# Autodesk Inventor assembly: Arduino_zlozenie
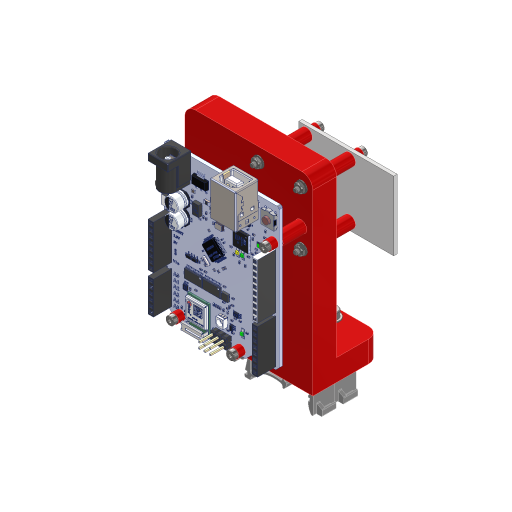
[picture p0: Inventor's stored thumbnail of the model, 512x512]
Saved by Autodesk Inventor 2024.3 (Build 283343000, 343)
## iProperties
Created: 2025-06-18
Part Number: Arduino_zlozenie
Document SubType Name: Assembly
Designer: MPA
Author: MPA
## Documents named in this file (13)
- C:\MPA - shortPath\magisterka\V3\Workspace\Arduino_zlozenie.iam
- C:\MPA - shortPath\magisterka\V3\Workspace\Zakupowe\arduino\Arduino UNO Wifi\Arduino UNO Wifi\Arduino UNO Wifi.ipt
- C:\MPA - shortPath\magisterka\V3\Workspace\MontazWszafie\Arduino-cz1.ipt
- C:\MPA - shortPath\magisterka\V3\Workspace\MontazWszafie\Arduino-cz2.ipt
- C:\MPA - shortPath\magisterka\V3\Workspace\MontazWszafie\2698103\2698103\NS_35_7.5_PERF_18X5.2_2000MM-Select.ipt
- C:\MPA - shortPath\magisterka\V3\Workspace\MontazWszafie\1201578_PHOENIX\1201578_PHOENIX\1201578_PHOENIX.ipt
- C:\MPA - shortPath\magisterka\V3\Workspace\MontazWszafie\Uchwyt_arduino.ipt
- C:\MPA - shortPath\magisterka\V3\Workspace\cc\en-US\Copy of DIN 912 - replaced by DIN EN ISO 4762\Copy of DIN 912 - M2 x 0,4 x 30 x 19.ipt
- C:\MPA - shortPath\magisterka\V3\Workspace\cc\en-US\DIN 125-1  A\DIN 125 - A 2,2.ipt
- C:\MPA - shortPath\magisterka\V3\Workspace\cc\en-US\DIN 934\DIN 934 - M2 x 0,4.ipt
- C:\MPA - shortPath\magisterka\V3\Workspace\cc\en-US\DIN 125-1  A\DIN 125 - A 3,2.ipt
- C:\MPA - shortPath\magisterka\V3\Workspace\cc\en-US\Copy of DIN 912 - replaced by DIN EN ISO 4762\Copy of DIN 912 - M3 x 0,5 x 16 x 14,75.ipt
- C:\MPA - shortPath\magisterka\V3\Workspace\DFR-08104.ipt
## Components (75 placed, 12 different names)
1. Arduino UNO Wifi:1 — Insert:1, Insert:2, Insert:3, Insert:4, Insert:5, Insert:6, Insert:7, Insert:8
2. Arduino-cz1:1 — Insert:2
3. Arduino-cz1:2 — Insert:3, Mate:5, Mate:7, Mate:9, Mate:11
4. Arduino-cz1:3 — Insert:4
5. Arduino-cz1:4 — Insert:1
6. Arduino-cz2:1 — Insert:5, Flush:9
7. Arduino-cz2:2 — Insert:6
8. Arduino-cz2:3 — Insert:7
9. Arduino-cz2:4 — Insert:8
10. NS_35_7.5_PERF_18X5.2_2000MM-Select:1 — Flush:4, Flush:5, Flush:6, Mate:2, Mate:3, Flush:11
11. 1201578_PHOENIX:1 — Flush:7, Flush:8, Mate:1, Mate:2
12. 1201578_PHOENIX:2 — Flush:7, Flush:8, Mate:1, Mate:3, Mate:20, Flush:10
13. Uchwyt_arduino:1 — Flush:9, Mate:4, Mate:6, Mate:8, Mate:10, Mate:12, Mate:13, Mate:14, Mate:15, Mate:16, Mate:17, Mate:18, Mate:19, Mate:20, Flush:10, Flush:11, Mate:21, Mate:22, Mate:23, Mate:24, Mate:25, Mate:26, Mate:27, Mate:28, Insert:33, Insert:34, Mate:29, Mate:30, Mate:31, Mate:33, Mate:35, Mate:37, Mate:39, Mate:41, Mate:43, Mate:45, Mate:47, Mate:48, Mate:49, Mate:50, Mate:51, Mate:52, Mate:53, Mate:54, Mate:55, Mate:56, Mate:57, Mate:58, Mate:59, Mate:60, Mate:61, Mate:62
14. Copy of DIN 912 - replaced by DIN EN ISO 4762 M2 x 30:1 — Mate:4, Mate:5
15. DIN 125-1 A A 2,2:1 — Mate:12, Mate:13, Insert:9
16. DIN 934 - replaced by DIN EN 24032/28673/28674 M2:1 — Insert:9
17. Copy of DIN 912 - replaced by DIN EN ISO 4762 M2 x 30:2 — Mate:6, Mate:7
18. Copy of DIN 912 - replaced by DIN EN ISO 4762 M2 x 30:3 — Mate:8, Mate:9
19. Copy of DIN 912 - replaced by DIN EN ISO 4762 M2 x 30:4 — Mate:10, Mate:11
20. DIN 125-1 A A 2,2:2 — Mate:14, Mate:15, Insert:10
21. DIN 125-1 A A 2,2:3 — Mate:16, Mate:17, Insert:11
22. DIN 125-1 A A 2,2:4 — Mate:18, Mate:19, Insert:12
23. DIN 934 - replaced by DIN EN 24032/28673/28674 M2:2 — Insert:10
24. DIN 934 - replaced by DIN EN 24032/28673/28674 M2:3 — Insert:11
25. DIN 934 - replaced by DIN EN 24032/28673/28674 M2:4 — Insert:12
26. DIN 125-1 A A 3,2:1 — Mate:21, Mate:22, Insert:13
27. Copy of DIN 912 - replaced by DIN EN ISO 4762 M3 x 16:1 — Insert:13
28. DIN 125-1 A A 3,2:2 — Mate:23, Mate:24, Insert:14
29. DIN 125-1 A A 3,2:3 — Mate:25, Mate:26, Insert:15
30. DIN 125-1 A A 3,2:4 — Mate:27, Mate:28, Insert:16
31. Copy of DIN 912 - replaced by DIN EN ISO 4762 M3 x 16:2 — Insert:14
32. Copy of DIN 912 - replaced by DIN EN ISO 4762 M3 x 16:3 — Insert:15
33. Copy of DIN 912 - replaced by DIN EN ISO 4762 M3 x 16:4 — Insert:16
34. Arduino-cz2:6 — Insert:17, Mate:30
35. Arduino-cz2:7 — Insert:19
36. Arduino-cz2:8 — Insert:18, Insert:33
37. Arduino-cz2:9 — Insert:20
38. DFR-08104:2 — Insert:17, Insert:18, Insert:19, Insert:20, Insert:21, Insert:22, Insert:23, Insert:24
39. Arduino-cz1:5 — Insert:21
40. Arduino-cz1:6 — Insert:23
41. Arduino-cz1:7 — Insert:24
42. Arduino-cz1:8 — Insert:22
43. Arduino-cz2:10 — Insert:34
44. Arduino-cz2:11
45. Arduino-cz2:12 — Mate:29
46. Arduino-cz2:13
47. DFR-08104:3
48. Arduino-cz1:9
49. Arduino-cz1:10
50. Arduino-cz1:11 — Mate:32, Mate:34, Mate:36, Mate:38, Mate:40, Mate:42, Mate:44, Mate:46
51. Arduino-cz1:12
52. Copy of DIN 912 - replaced by DIN EN ISO 4762 M2 x 30:5 — Mate:31, Mate:32
53. DIN 125-1 A A 2,2:5 — Mate:47, Mate:48, Insert:35
54. DIN 934 - replaced by DIN EN 24032/28673/28674 M2:5 — Insert:35
55. Copy of DIN 912 - replaced by DIN EN ISO 4762 M2 x 30:6 — Mate:33, Mate:34
56. Copy of DIN 912 - replaced by DIN EN ISO 4762 M2 x 30:7 — Mate:35, Mate:36
57. Copy of DIN 912 - replaced by DIN EN ISO 4762 M2 x 30:8 — Mate:37, Mate:38
58. Copy of DIN 912 - replaced by DIN EN ISO 4762 M2 x 30:9 — Mate:39, Mate:40
59. Copy of DIN 912 - replaced by DIN EN ISO 4762 M2 x 30:10 — Mate:41, Mate:42
60. Copy of DIN 912 - replaced by DIN EN ISO 4762 M2 x 30:11 — Mate:43, Mate:44
61. Copy of DIN 912 - replaced by DIN EN ISO 4762 M2 x 30:12 — Mate:45, Mate:46
62. DIN 125-1 A A 2,2:6 — Mate:49, Mate:50, Insert:36
63. DIN 125-1 A A 2,2:7 — Mate:51, Mate:52, Insert:37
64. DIN 125-1 A A 2,2:8 — Mate:53, Mate:54, Insert:38
65. DIN 125-1 A A 2,2:9 — Mate:55, Mate:56, Insert:39
66. DIN 125-1 A A 2,2:10 — Mate:57, Mate:58, Insert:40
67. DIN 125-1 A A 2,2:11 — Mate:59, Mate:60, Insert:41
68. DIN 125-1 A A 2,2:12 — Mate:61, Mate:62, Insert:42
69. DIN 934 - replaced by DIN EN 24032/28673/28674 M2:6 — Insert:36
70. DIN 934 - replaced by DIN EN 24032/28673/28674 M2:7 — Insert:37
71. DIN 934 - replaced by DIN EN 24032/28673/28674 M2:8 — Insert:38
72. DIN 934 - replaced by DIN EN 24032/28673/28674 M2:9 — Insert:39
73. DIN 934 - replaced by DIN EN 24032/28673/28674 M2:10 — Insert:40
74. DIN 934 - replaced by DIN EN 24032/28673/28674 M2:11 — Insert:41
75. DIN 934 - replaced by DIN EN 24032/28673/28674 M2:12 — Insert:42
## Relationships (112: Mate 62, Insert 42, Flush 8)
- Insert:1: Arduino UNO Wifi:1 ↔ Arduino-cz1:4
- Insert:2: Arduino UNO Wifi:1 ↔ Arduino-cz1:1
- Insert:3: Arduino UNO Wifi:1 ↔ Arduino-cz1:2
- Insert:4: Arduino UNO Wifi:1 ↔ Arduino-cz1:3
- Insert:5: Arduino UNO Wifi:1 ↔ Arduino-cz2:1
- Insert:6: Arduino UNO Wifi:1 ↔ Arduino-cz2:2
- Insert:7: Arduino UNO Wifi:1 ↔ Arduino-cz2:3
- Insert:8: Arduino UNO Wifi:1 ↔ Arduino-cz2:4
- Flush:4: NS_35_7.5_PERF_18X5.2_2000MM-Select:1
- Flush:5: NS_35_7.5_PERF_18X5.2_2000MM-Select:1
- Flush:6: NS_35_7.5_PERF_18X5.2_2000MM-Select:1
- Flush:7: 1201578_PHOENIX:1 ↔ 1201578_PHOENIX:2
- Flush:8: 1201578_PHOENIX:1 ↔ 1201578_PHOENIX:2
- Mate:1: 1201578_PHOENIX:1 ↔ 1201578_PHOENIX:2
- Mate:2: NS_35_7.5_PERF_18X5.2_2000MM-Select:1 ↔ 1201578_PHOENIX:1
- Mate:3: NS_35_7.5_PERF_18X5.2_2000MM-Select:1 ↔ 1201578_PHOENIX:2
- Flush:9: Arduino-cz2:1 ↔ Uchwyt_arduino:1
- Mate:4: Uchwyt_arduino:1 ↔ Copy of DIN 912 - replaced by DIN EN ISO 4762 M2 x 30:1
- Mate:5: Arduino-cz1:2 ↔ Copy of DIN 912 - replaced by DIN EN ISO 4762 M2 x 30:1
- Mate:6: Uchwyt_arduino:1 ↔ Copy of DIN 912 - replaced by DIN EN ISO 4762 M2 x 30:2
- Mate:7: Arduino-cz1:2 ↔ Copy of DIN 912 - replaced by DIN EN ISO 4762 M2 x 30:2
- Mate:8: Uchwyt_arduino:1 ↔ Copy of DIN 912 - replaced by DIN EN ISO 4762 M2 x 30:3
- Mate:9: Arduino-cz1:2 ↔ Copy of DIN 912 - replaced by DIN EN ISO 4762 M2 x 30:3
- Mate:10: Uchwyt_arduino:1 ↔ Copy of DIN 912 - replaced by DIN EN ISO 4762 M2 x 30:4
- Mate:11: Arduino-cz1:2 ↔ Copy of DIN 912 - replaced by DIN EN ISO 4762 M2 x 30:4
- Mate:12: Uchwyt_arduino:1 ↔ DIN 125-1 A A 2,2:1
- Mate:13: Uchwyt_arduino:1 ↔ DIN 125-1 A A 2,2:1
- Mate:14: Uchwyt_arduino:1 ↔ DIN 125-1 A A 2,2:2
- Mate:15: Uchwyt_arduino:1 ↔ DIN 125-1 A A 2,2:2
- Mate:16: Uchwyt_arduino:1 ↔ DIN 125-1 A A 2,2:3
- Mate:17: Uchwyt_arduino:1 ↔ DIN 125-1 A A 2,2:3
- Mate:18: Uchwyt_arduino:1 ↔ DIN 125-1 A A 2,2:4
- Mate:19: Uchwyt_arduino:1 ↔ DIN 125-1 A A 2,2:4
- Insert:9: DIN 125-1 A A 2,2:1 ↔ DIN 934 - replaced by DIN EN 24032/28673/28674 M2:1
- Insert:10: DIN 125-1 A A 2,2:2 ↔ DIN 934 - replaced by DIN EN 24032/28673/28674 M2:2
- Insert:11: DIN 125-1 A A 2,2:3 ↔ DIN 934 - replaced by DIN EN 24032/28673/28674 M2:3
- Insert:12: DIN 125-1 A A 2,2:4 ↔ DIN 934 - replaced by DIN EN 24032/28673/28674 M2:4
- Mate:20: 1201578_PHOENIX:2 ↔ Uchwyt_arduino:1
- Flush:10: 1201578_PHOENIX:2 ↔ Uchwyt_arduino:1
- Flush:11 (-12.2 mm): NS_35_7.5_PERF_18X5.2_2000MM-Select:1 ↔ Uchwyt_arduino:1
- Mate:21: Uchwyt_arduino:1 ↔ DIN 125-1 A A 3,2:1
- Mate:22: Uchwyt_arduino:1 ↔ DIN 125-1 A A 3,2:1
- Mate:23: Uchwyt_arduino:1 ↔ DIN 125-1 A A 3,2:2
- Mate:24: Uchwyt_arduino:1 ↔ DIN 125-1 A A 3,2:2
- Mate:25: Uchwyt_arduino:1 ↔ DIN 125-1 A A 3,2:3
- Mate:26: Uchwyt_arduino:1 ↔ DIN 125-1 A A 3,2:3
- Mate:27: Uchwyt_arduino:1 ↔ DIN 125-1 A A 3,2:4
- Mate:28: Uchwyt_arduino:1 ↔ DIN 125-1 A A 3,2:4
- Insert:13: DIN 125-1 A A 3,2:1 ↔ Copy of DIN 912 - replaced by DIN EN ISO 4762 M3 x 16:1
- Insert:14: DIN 125-1 A A 3,2:2 ↔ Copy of DIN 912 - replaced by DIN EN ISO 4762 M3 x 16:2
- Insert:15: DIN 125-1 A A 3,2:3 ↔ Copy of DIN 912 - replaced by DIN EN ISO 4762 M3 x 16:3
- Insert:16: DIN 125-1 A A 3,2:4 ↔ Copy of DIN 912 - replaced by DIN EN ISO 4762 M3 x 16:4
- Insert:17: Arduino-cz2:6 ↔ DFR-08104:2
- Insert:18: Arduino-cz2:8 ↔ DFR-08104:2
- Insert:19: Arduino-cz2:7 ↔ DFR-08104:2
- Insert:20: Arduino-cz2:9 ↔ DFR-08104:2
- Insert:21: DFR-08104:2 ↔ Arduino-cz1:5
- Insert:22: DFR-08104:2 ↔ Arduino-cz1:8
- Insert:23: DFR-08104:2 ↔ Arduino-cz1:6
- Insert:24: DFR-08104:2 ↔ Arduino-cz1:7
- [Insert]: Arduino-cz2:10 ↔ DFR-08104:3
- [Insert]: Arduino-cz2:12 ↔ DFR-08104:3
- [Insert]: Arduino-cz2:11 ↔ DFR-08104:3
- [Insert]: Arduino-cz2:13 ↔ DFR-08104:3
- [Insert]: DFR-08104:3 ↔ Arduino-cz1:9
- [Insert]: DFR-08104:3 ↔ Arduino-cz1:12
- [Insert]: DFR-08104:3 ↔ Arduino-cz1:10
- [Insert]: DFR-08104:3 ↔ Arduino-cz1:11
- Insert:33: Uchwyt_arduino:1 ↔ Arduino-cz2:8
- Insert:34: Uchwyt_arduino:1 ↔ Arduino-cz2:10
- Mate:29: Uchwyt_arduino:1 ↔ Arduino-cz2:12
- Mate:30: Uchwyt_arduino:1 ↔ Arduino-cz2:6
- Mate:31: Uchwyt_arduino:1 ↔ Copy of DIN 912 - replaced by DIN EN ISO 4762 M2 x 30:5
- Mate:32: Arduino-cz1:11 ↔ Copy of DIN 912 - replaced by DIN EN ISO 4762 M2 x 30:5
- Mate:33: Uchwyt_arduino:1 ↔ Copy of DIN 912 - replaced by DIN EN ISO 4762 M2 x 30:6
- Mate:34: Arduino-cz1:11 ↔ Copy of DIN 912 - replaced by DIN EN ISO 4762 M2 x 30:6
- Mate:35: Uchwyt_arduino:1 ↔ Copy of DIN 912 - replaced by DIN EN ISO 4762 M2 x 30:7
- Mate:36: Arduino-cz1:11 ↔ Copy of DIN 912 - replaced by DIN EN ISO 4762 M2 x 30:7
- Mate:37: Uchwyt_arduino:1 ↔ Copy of DIN 912 - replaced by DIN EN ISO 4762 M2 x 30:8
- Mate:38: Arduino-cz1:11 ↔ Copy of DIN 912 - replaced by DIN EN ISO 4762 M2 x 30:8
- Mate:39: Uchwyt_arduino:1 ↔ Copy of DIN 912 - replaced by DIN EN ISO 4762 M2 x 30:9
- Mate:40: Arduino-cz1:11 ↔ Copy of DIN 912 - replaced by DIN EN ISO 4762 M2 x 30:9
- Mate:41: Uchwyt_arduino:1 ↔ Copy of DIN 912 - replaced by DIN EN ISO 4762 M2 x 30:10
- Mate:42: Arduino-cz1:11 ↔ Copy of DIN 912 - replaced by DIN EN ISO 4762 M2 x 30:10
- Mate:43: Uchwyt_arduino:1 ↔ Copy of DIN 912 - replaced by DIN EN ISO 4762 M2 x 30:11
- Mate:44: Arduino-cz1:11 ↔ Copy of DIN 912 - replaced by DIN EN ISO 4762 M2 x 30:11
- Mate:45: Uchwyt_arduino:1 ↔ Copy of DIN 912 - replaced by DIN EN ISO 4762 M2 x 30:12
- Mate:46: Arduino-cz1:11 ↔ Copy of DIN 912 - replaced by DIN EN ISO 4762 M2 x 30:12
- Mate:47: Uchwyt_arduino:1 ↔ DIN 125-1 A A 2,2:5
- Mate:48: Uchwyt_arduino:1 ↔ DIN 125-1 A A 2,2:5
- Mate:49: Uchwyt_arduino:1 ↔ DIN 125-1 A A 2,2:6
- Mate:50: Uchwyt_arduino:1 ↔ DIN 125-1 A A 2,2:6
- Mate:51: Uchwyt_arduino:1 ↔ DIN 125-1 A A 2,2:7
- Mate:52: Uchwyt_arduino:1 ↔ DIN 125-1 A A 2,2:7
- Mate:53: Uchwyt_arduino:1 ↔ DIN 125-1 A A 2,2:8
- Mate:54: Uchwyt_arduino:1 ↔ DIN 125-1 A A 2,2:8
- Mate:55: Uchwyt_arduino:1 ↔ DIN 125-1 A A 2,2:9
- Mate:56: Uchwyt_arduino:1 ↔ DIN 125-1 A A 2,2:9
- Mate:57: Uchwyt_arduino:1 ↔ DIN 125-1 A A 2,2:10
- Mate:58: Uchwyt_arduino:1 ↔ DIN 125-1 A A 2,2:10
- Mate:59: Uchwyt_arduino:1 ↔ DIN 125-1 A A 2,2:11
- Mate:60: Uchwyt_arduino:1 ↔ DIN 125-1 A A 2,2:11
- Mate:61: Uchwyt_arduino:1 ↔ DIN 125-1 A A 2,2:12
- Mate:62: Uchwyt_arduino:1 ↔ DIN 125-1 A A 2,2:12
- Insert:35: DIN 125-1 A A 2,2:5 ↔ DIN 934 - replaced by DIN EN 24032/28673/28674 M2:5
- Insert:36: DIN 125-1 A A 2,2:6 ↔ DIN 934 - replaced by DIN EN 24032/28673/28674 M2:6
- Insert:37: DIN 125-1 A A 2,2:7 ↔ DIN 934 - replaced by DIN EN 24032/28673/28674 M2:7
- Insert:38: DIN 125-1 A A 2,2:8 ↔ DIN 934 - replaced by DIN EN 24032/28673/28674 M2:8
- Insert:39: DIN 125-1 A A 2,2:9 ↔ DIN 934 - replaced by DIN EN 24032/28673/28674 M2:9
- Insert:40: DIN 125-1 A A 2,2:10 ↔ DIN 934 - replaced by DIN EN 24032/28673/28674 M2:10
- Insert:41: DIN 125-1 A A 2,2:11 ↔ DIN 934 - replaced by DIN EN 24032/28673/28674 M2:11
- Insert:42: DIN 125-1 A A 2,2:12 ↔ DIN 934 - replaced by DIN EN 24032/28673/28674 M2:12
## Named parameters: d146_d139 = 0 mm, d147_d138 = 0 mm, d148_d140 = 0 mm, d149_d141 = 0 mm, d150_d142 = 0 mm, d151_d144 = 0 mm, d152_d145 = 0 mm, d153_d143 = 0 mm
